# Autodesk Inventor assembly: 3.25 omni 60t
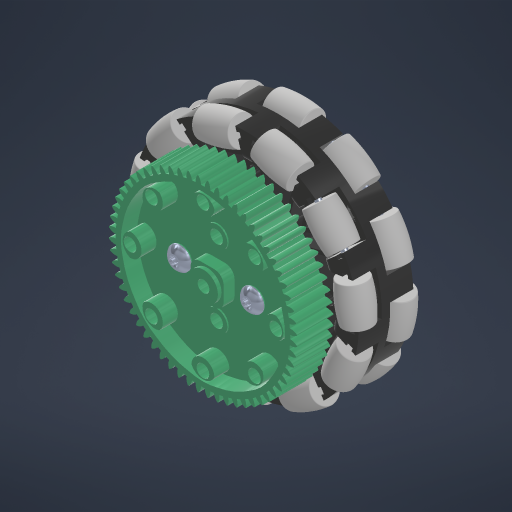
[picture p0: Inventor's stored thumbnail of the model, 512x512]
Saved by Autodesk Inventor 2023 (Build 270158000, 158)
## iProperties
Created: 2023-03-19
Part Number: 3.25 omni 60t
Document SubType Name: Assembly
Designer: Main Account
Author: Main Account
## Documents named in this file (12)
- D:\Documents\Inventor\VEX\Custom Library\3.25 omni 60t.iam
- D:\Documents\Inventor\VEX\Library Backup\Library 1.4\Motion\Wheels\Omni Wheel\3.25 Omni AS, No Insert.iam
- D:\Documents\Inventor\VEX\Library Backup\Library 1.4\Motion\Wheels\Omni Wheel.iam
- D:\Documents\Inventor\VEX\Library Backup\Library 1.4\Motion\Gears\HS Gear\Old Gears\HS 60T Gear, No Insert.ipt
- D:\Documents\Inventor\VEX\Library Backup\Library 1.4\Structure\Hardware\Screw Steel - Star\SScrew Star Smooth 1.250.ipt
- D:\Documents\Inventor\VEX\Library Backup\Library 1.4\Structure\Hardware\Screw Steel - Star.ipt
- D:\Documents\Inventor\VEX\Library Backup\Library 1.4\Motion\Spacers\Spacer Nylon .375 OD.ipt
- D:\Documents\Inventor\VEX\Library Backup\Library 1.4\Motion\Spacers\Washer Steel\SWasher .375 OD x .031250.ipt
- D:\Documents\Inventor\VEX\Library Backup\Library 1.4\Motion\Spacers\Washer Steel.ipt
- D:\Documents\Inventor\VEX\Library Backup\Library 1.4\Structure\Hardware\Nut Thin Nylock.ipt
- D:\Documents\Inventor\VEX\Library Backup\Library 1.4\Motion\Spacers\Spacer Nylon .375 OD\NSpacer .375 OD x .375.ipt
- D:\Documents\Inventor\VEX\Library Backup\Library 1.4\Motion\Insert Circle Green.ipt
## Components (12 placed, 7 different names)
1. 3.25 Omni AS, No Insert:1 [sub-assembly] — Mate:1, Insert:4, Insert:8, Insert:9, Insert:11
2. HS 60T Gear, No Insert:1 — Mate:1, Insert:1, Insert:3, Insert:6, Insert:7, Insert:10
3. SScrew Star Smooth 1.250:1 — Insert:1
4. NSpacer .375 OD x .375:1 — Insert:2
5. SWasher .375 OD x .031250:1 — Insert:2, Insert:3
6. Nut Thin Nylock:1 — Insert:4
7. SScrew Star Smooth 1.250:2 — Insert:6
8. NSpacer .375 OD x .375:2 — Insert:9
9. SWasher .375 OD x .031250:2 — Insert:7
10. Nut Thin Nylock:2 — Insert:8
11. Insert Circle Green:1 — Insert:10
12. Insert Circle Green:2 — Insert:11
## Relationships (12: Insert 11, Mate 1)
- Mate:1: 3.25 Omni AS, No Insert:1 ↔ HS 60T Gear, No Insert:1
- Insert:1: HS 60T Gear, No Insert:1 ↔ SScrew Star Smooth 1.250:1
- Insert:2: NSpacer .375 OD x .375:1 ↔ SWasher .375 OD x .031250:1
- Insert:3: HS 60T Gear, No Insert:1 ↔ SWasher .375 OD x .031250:1
- Insert:4: 3.25 Omni AS, No Insert:1 ↔ Nut Thin Nylock:1
- [Insert]: NSpacer .375 OD x .375:2 ↔ SWasher .375 OD x .031250:2
- Insert:6: HS 60T Gear, No Insert:1 ↔ SScrew Star Smooth 1.250:2
- Insert:7: HS 60T Gear, No Insert:1 ↔ SWasher .375 OD x .031250:2
- Insert:8: 3.25 Omni AS, No Insert:1 ↔ Nut Thin Nylock:2
- Insert:9: 3.25 Omni AS, No Insert:1 ↔ NSpacer .375 OD x .375:2
- Insert:10: HS 60T Gear, No Insert:1 ↔ Insert Circle Green:1
- Insert:11: 3.25 Omni AS, No Insert:1 ↔ Insert Circle Green:2
## Named parameters: d5_d2 = 0 mm
